# Autodesk Inventor assembly: 1310 ASY GBK long wall shield 4
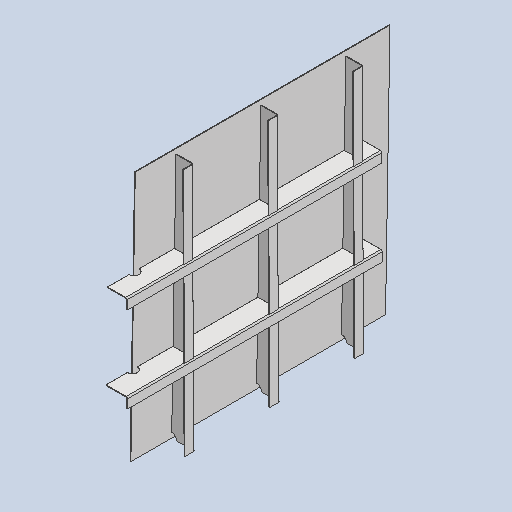
[picture p0: Inventor's stored thumbnail of the model, 512x512]
Saved by Autodesk Inventor 2026.2 (Build 302298000, 298)
## iProperties
Created: 2026-05-07
Part Number: 1310 ASY GBK long wall shield 4
Document SubType Name: Assembly
Designer: pokla
Mass: 107756 g
Surface Area: 69611.7 cm^2
Volume: 13726.9 cm^3
Density: 7.85 g/cm^3
Author: admin
## Documents named in this file (6)
- C:\Users\admin\Documents\Inventor\GBK-Gubkinskiy\07 ASY GBK wall shield 1.3.1.iam
- C:\Users\admin\Documents\Inventor\GBK-Gubkinskiy\07.1 GBK shield.ipt
- C:\Users\admin\Documents\Inventor\GBK-Gubkinskiy\07.2 GBK rib.ipt
- C:\Users\admin\Documents\Inventor\GBK-Gubkinskiy\0371 GBK stringer 7.ipt
- C:\Users\admin\Documents\Inventor\GBK-Gubkinskiy\0372 GBK stringer 8.ipt
- C:\Users\admin\Documents\Inventor\GBK-Gubkinskiy\01.2 GBK main rib.ipt
## Components (6 placed, 4 different names)
1. 0371 GBK stringer 7:1
2. 0372 GBK stringer 8:1
3. 07.1 GBK shield:1
4. 07.2 GBK rib:1
5. 07.2 GBK rib:2
6. 07.2 GBK rib:3
## Component patterns: (3 elements, first: 07.2 GBK rib:1)
## Relationships (5: Mate 2, WeldJoint 2, Flush 1)
- [Flush] (254 mm): 07.1 GBK shield:1 ↔ 07.2 GBK rib:1
- [Mate]: 07.1 GBK shield:1 ↔ 07.2 GBK rib:1
- [Mate]: 07.1 GBK shield:1 ↔ 07.2 GBK rib:1
- [WeldJoint] (4 mm): 0371 GBK stringer 7:1 ↔ 07.2 GBK rib:1
- [WeldJoint] (4 mm): 0372 GBK stringer 8:1 ↔ 07.2 GBK rib:1
## Named parameters: Шаг_шпангоутов = 496.66667 mm
